# Autodesk Inventor assembly: Ares 2_0
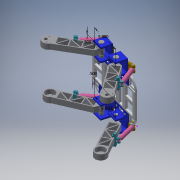
[picture p0: Inventor's stored thumbnail of the model, 180x180]
Saved by Autodesk Inventor 2018.2 (Build 222227000, 227)
## iProperties
Created: 2018-03-23
Part Number: Ares 2_0
Document SubType Name: Assembly
Designer: MIABo
Author: MIABo
## Documents named in this file (16)
- C:\Users\MIABo\OneDrive\Documents\GitHub\Ares\3D Model Files\Ares 2_0.iam
- C:\Users\MIABo\OneDrive\Documents\GitHub\Ares\3D Model Files\Frame 2.1.ipt
- C:\Users\MIABo\OneDrive\Documents\GitHub\Ares\3D Model Files\Suspension Frame 3.0.ipt
- C:\Users\MIABo\OneDrive\Documents\GitHub\Ares\3D Model Files\Frame mount rivet.ipt
- C:\Users\MIABo\OneDrive\Documents\GitHub\Ares\3D Model Files\Leg Mount Rivet.ipt
- C:\Users\MIABo\OneDrive\Documents\GitHub\Ares\3D Model Files\Leg Spacer.ipt
- C:\Users\MIABo\OneDrive\Documents\GitHub\Ares\3D Model Files\Ultrasonic MoUnt.ipt
- C:\Users\MIABo\OneDrive\Documents\GitHub\Ares\3D Model Files\Ares 2_0\Design Accelerator\Clevis Pin Connection1.iam
- C:\Users\MIABo\OneDrive\Documents\GitHub\Ares\3D Model Files\Ares 2_0\Design Accelerator\Clevis Pin Connection2.iam
- C:\Users\MIABo\OneDrive\Documents\GitHub\Ares\3D Model Files\Upper_Spring_Hanger.ipt
- C:\Users\MIABo\OneDrive\Documents\GitHub\Ares\3D Model Files\leg 3.0.ipt
- C:\Users\MIABo\OneDrive\Documents\GitHub\Ares\3D Model Files\SpringPin.ipt
- C:\Users\MIABo\OneDrive\Documents\GitHub\Ares\3D Model Files\MockShock2.ipt
- C:\Users\MIABo\OneDrive\Documents\GitHub\Ares\3D Model Files\LowerSpringMountRearBracket.ipt
- C:\Users\MIABo\OneDrive\Documents\GitHub\Ares\3D Model Files\LowerSpringMountFront.ipt
- C:\Users\MIABo\OneDrive\Documents\GitHub\Ares\3D Model Files\Upper_Spring_Hanger2.ipt
## Components (56 placed, 14 different names)
1. Frame 2.1:1 — Mate:1, Mate:2, Mate:3, Mate:4, Mate:5, Mate:6, Mate:8, Mate:9, Mate:10, Mate:11, Mate:13, Mate:14, Flush:1
2. Suspension Frame 3.0:1 — Mate:1, Mate:2, Mate:4, Insert:5, Insert:6, Insert:9, Insert:16, Insert:22, Mate:31, Tangent:10, Tangent:11
3. Suspension Frame 3.0:2 — Mate:3, Mate:5, Mate:6, Insert:7, Insert:8, Insert:10, Insert:15, Insert:21, Mate:17, Insert:25, Insert:26
4. Suspension Frame 3.0:3 — Mate:8, Mate:9, Mate:10, Mate:12, Insert:2, Insert:3, Insert:11, Insert:13, Insert:20, Mate:16, Insert:29, Insert:30
5. Suspension Frame 3.0:4 — Mate:11, Mate:12, Mate:13, Insert:1, Insert:4, Insert:12, Insert:14, Mate:32, Tangent:13, Tangent:14
6. Frame mount rivet:1 — Insert:8
7. Frame mount rivet:2 — Insert:7
8. Frame mount rivet:3 — Insert:6
9. Frame mount rivet:4 — Insert:2
10. Frame mount rivet:5 — Insert:3
11. Frame mount rivet:6 — Insert:4
12. Frame mount rivet:7 — Insert:5
13. Frame mount rivet:8 — Insert:1
14. Leg Mount Rivet:1 — Insert:9
15. Leg Mount Rivet:2 — Insert:10
16. Leg Mount Rivet:3 — Insert:11
17. Leg Mount Rivet:4 — Insert:12
18. Leg Spacer:1 — Insert:22
19. Leg Spacer:2 — Insert:21
20. Leg Spacer:3 — Insert:20, Insert:33
21. Leg Spacer:4 — Insert:13
22. Leg Spacer:5 — Insert:14, Insert:34
23. Leg Spacer:6 — Insert:15, Insert:32
24. Leg Spacer:7 — Insert:16, Insert:31
25. Leg Spacer:8
26. Ultrasonic MoUnt:1 — Mate:14, Flush:1
27. Clevis Pin Connection:1 [sub-assembly]
28. Clevis Pin Connection:2 [sub-assembly]
29. Upper_Spring_Hanger:2 — Mate:16, Insert:29, Insert:30, Insert:37, Insert:38
30. Upper_Spring_Hanger:3 — Mate:17, Insert:25, Insert:26, Insert:45, Insert:46
31. leg 3.0:1 — Insert:31, Mate:27, Mate:28, Mate:29, Mate:36
32. leg 3.0:2 — Insert:34, Mate:22, Mate:23, Mate:34
33. leg 3.0:3 — Insert:33, Mate:19, Mate:20, Mate:35
34. leg 3.0:4 — Insert:32, Mate:25, Mate:26, Mate:30, Mate:33
35. SpringPin:1 — Insert:38
36. SpringPin:2 — Insert:39, Mate:21
37. SpringPin:3 — Insert:49
38. SpringPin:4 — Insert:47, Tangent:8
39. SpringPin:5 — Insert:50
40. SpringPin:6 — Insert:45
41. SpringPin:7 — Insert:48, Tangent:15
42. SpringPin:8 — Insert:42, Tangent:16
43. MockShock2:1 — Insert:37, Mate:21
44. MockShock2:3 — Insert:46, Tangent:8
45. LowerSpringMountRearBracket:1 — Mate:27, Mate:28, Tangent:4, Tangent:5, Mate:36
46. LowerSpringMountRearBracket:2 — Mate:22, Mate:23, Mate:24, Tangent:1, Tangent:2, Mate:34
47. LowerSpringMountRearBracket:3 — Mate:25, Mate:26, Tangent:6, Tangent:7, Mate:33
48. LowerSpringMountRearBracket:4 — Mate:19, Mate:20, Insert:35, Insert:36, Mate:35
49. LowerSpringMountFront:1 — Mate:24, Tangent:1, Tangent:2, Insert:42
50. LowerSpringMountFront:2 — Insert:47, Mate:30, Tangent:6, Tangent:7
51. LowerSpringMountFront:3 — Insert:48, Mate:29, Tangent:4, Tangent:5
52. LowerSpringMountFront:4 — Insert:35, Insert:36, Insert:39
53. Upper_Spring_Hanger2:1 — Mate:32, Tangent:13, Tangent:14, Insert:50, Insert:52
54. Upper_Spring_Hanger2:2 — Mate:31, Tangent:10, Tangent:11, Insert:49, Insert:51
55. MockShock2:5 — Insert:52, Tangent:16
56. MockShock2:6 — Insert:51, Tangent:15
## Relationships (88: Insert 41, Mate 33, Tangent 13, Flush 1)
- Mate:1: Frame 2.1:1 ↔ Suspension Frame 3.0:1
- Mate:2: Frame 2.1:1 ↔ Suspension Frame 3.0:1
- Mate:3: Frame 2.1:1 ↔ Suspension Frame 3.0:2
- Mate:4: Frame 2.1:1 ↔ Suspension Frame 3.0:1
- Mate:5: Frame 2.1:1 ↔ Suspension Frame 3.0:2
- Mate:6: Frame 2.1:1 ↔ Suspension Frame 3.0:2
- Mate:8: Frame 2.1:1 ↔ Suspension Frame 3.0:3
- Mate:9: Frame 2.1:1 ↔ Suspension Frame 3.0:3
- Mate:10: Frame 2.1:1 ↔ Suspension Frame 3.0:3
- Mate:11: Frame 2.1:1 ↔ Suspension Frame 3.0:4
- Mate:12: Suspension Frame 3.0:3 ↔ Suspension Frame 3.0:4
- Mate:13: Frame 2.1:1 ↔ Suspension Frame 3.0:4
- Insert:1 (-15.24 mm): Suspension Frame 3.0:4 ↔ Frame mount rivet:8
- Insert:2 (-15.24 mm): Suspension Frame 3.0:3 ↔ Frame mount rivet:4
- Insert:3 (-15.24 mm): Suspension Frame 3.0:3 ↔ Frame mount rivet:5
- Insert:4 (-15.24 mm): Suspension Frame 3.0:4 ↔ Frame mount rivet:6
- Insert:5 (-15.24 mm): Suspension Frame 3.0:1 ↔ Frame mount rivet:7
- Insert:6 (-15.24 mm): Suspension Frame 3.0:1 ↔ Frame mount rivet:3
- Insert:7 (-15.24 mm): Suspension Frame 3.0:2 ↔ Frame mount rivet:2
- Insert:8 (-15.24 mm): Suspension Frame 3.0:2 ↔ Frame mount rivet:1
- Insert:9: Suspension Frame 3.0:1 ↔ Leg Mount Rivet:1
- Insert:10: Suspension Frame 3.0:2 ↔ Leg Mount Rivet:2
- Insert:11: Suspension Frame 3.0:3 ↔ Leg Mount Rivet:3
- Insert:12: Suspension Frame 3.0:4 ↔ Leg Mount Rivet:4
- Insert:13: Suspension Frame 3.0:3 ↔ Leg Spacer:4
- Insert:14: Suspension Frame 3.0:4 ↔ Leg Spacer:5
- Insert:15: Suspension Frame 3.0:2 ↔ Leg Spacer:6
- Insert:16: Suspension Frame 3.0:1 ↔ Leg Spacer:7
- Insert:20: Suspension Frame 3.0:3 ↔ Leg Spacer:3
- Insert:21: Suspension Frame 3.0:2 ↔ Leg Spacer:2
- Insert:22: Suspension Frame 3.0:1 ↔ Leg Spacer:1
- Mate:14: Frame 2.1:1 ↔ Ultrasonic MoUnt:1
- Flush:1: Frame 2.1:1 ↔ Ultrasonic MoUnt:1
- Mate:16: Suspension Frame 3.0:3 ↔ Upper_Spring_Hanger:2
- Mate:17: Suspension Frame 3.0:2 ↔ Upper_Spring_Hanger:3
- Insert:25: Suspension Frame 3.0:2 ↔ Upper_Spring_Hanger:3
- Insert:26: Suspension Frame 3.0:2 ↔ Upper_Spring_Hanger:3
- Insert:29: Suspension Frame 3.0:3 ↔ Upper_Spring_Hanger:2
- Insert:30: Suspension Frame 3.0:3 ↔ Upper_Spring_Hanger:2
- Insert:31: Leg Spacer:7 ↔ leg 3.0:1
- Insert:32: Leg Spacer:6 ↔ leg 3.0:4
- Insert:33: Leg Spacer:3 ↔ leg 3.0:3
- Insert:34: Leg Spacer:5 ↔ leg 3.0:2
- Mate:19: leg 3.0:3 ↔ LowerSpringMountRearBracket:4
- Mate:20: leg 3.0:3 ↔ LowerSpringMountRearBracket:4
- Insert:35: LowerSpringMountRearBracket:4 ↔ LowerSpringMountFront:4
- Insert:36: LowerSpringMountRearBracket:4 ↔ LowerSpringMountFront:4
- Insert:37: Upper_Spring_Hanger:2 ↔ MockShock2:1
- Insert:38: Upper_Spring_Hanger:2 ↔ SpringPin:1
- Insert:39: SpringPin:2 ↔ LowerSpringMountFront:4
- Mate:21: SpringPin:2 ↔ MockShock2:1
- Mate:22: leg 3.0:2 ↔ LowerSpringMountRearBracket:2
- Mate:23: leg 3.0:2 ↔ LowerSpringMountRearBracket:2
- Mate:24: LowerSpringMountRearBracket:2 ↔ LowerSpringMountFront:1
- Tangent:1: LowerSpringMountRearBracket:2 ↔ LowerSpringMountFront:1
- Tangent:2: LowerSpringMountRearBracket:2 ↔ LowerSpringMountFront:1
- Insert:42: SpringPin:8 ↔ LowerSpringMountFront:1
- Insert:45: Upper_Spring_Hanger:3 ↔ SpringPin:6
- Insert:46: Upper_Spring_Hanger:3 ↔ MockShock2:3
- Mate:25: leg 3.0:4 ↔ LowerSpringMountRearBracket:3
- Mate:26: leg 3.0:4 ↔ LowerSpringMountRearBracket:3
- Mate:27: leg 3.0:1 ↔ LowerSpringMountRearBracket:1
- Mate:28: leg 3.0:1 ↔ LowerSpringMountRearBracket:1
- Insert:47: SpringPin:4 ↔ LowerSpringMountFront:2
- Insert:48: SpringPin:7 ↔ LowerSpringMountFront:3
- Mate:29: leg 3.0:1 ↔ LowerSpringMountFront:3
- Tangent:4: LowerSpringMountRearBracket:1 ↔ LowerSpringMountFront:3
- Tangent:5: LowerSpringMountRearBracket:1 ↔ LowerSpringMountFront:3
- Mate:30: leg 3.0:4 ↔ LowerSpringMountFront:2
- Tangent:6: LowerSpringMountRearBracket:3 ↔ LowerSpringMountFront:2
- Tangent:7: LowerSpringMountRearBracket:3 ↔ LowerSpringMountFront:2
- Tangent:8: SpringPin:4 ↔ MockShock2:3
- Mate:31: Suspension Frame 3.0:1 ↔ Upper_Spring_Hanger2:2
- Tangent:10: Suspension Frame 3.0:1 ↔ Upper_Spring_Hanger2:2
- Tangent:11: Suspension Frame 3.0:1 ↔ Upper_Spring_Hanger2:2
- Insert:49: SpringPin:3 ↔ Upper_Spring_Hanger2:2
- Mate:32: Suspension Frame 3.0:4 ↔ Upper_Spring_Hanger2:1
- Tangent:13: Suspension Frame 3.0:4 ↔ Upper_Spring_Hanger2:1
- Tangent:14: Suspension Frame 3.0:4 ↔ Upper_Spring_Hanger2:1
- Insert:50: SpringPin:5 ↔ Upper_Spring_Hanger2:1
- Insert:51: Upper_Spring_Hanger2:2 ↔ MockShock2:6
- Tangent:15: SpringPin:7 ↔ MockShock2:6
- Insert:52: Upper_Spring_Hanger2:1 ↔ MockShock2:5
- Tangent:16: SpringPin:8 ↔ MockShock2:5
- Mate:33: leg 3.0:4 ↔ LowerSpringMountRearBracket:3
- Mate:34: leg 3.0:2 ↔ LowerSpringMountRearBracket:2
- Mate:35: leg 3.0:3 ↔ LowerSpringMountRearBracket:4
- Mate:36: leg 3.0:1 ↔ LowerSpringMountRearBracket:1
